# Autodesk Inventor assembly: Assembly3
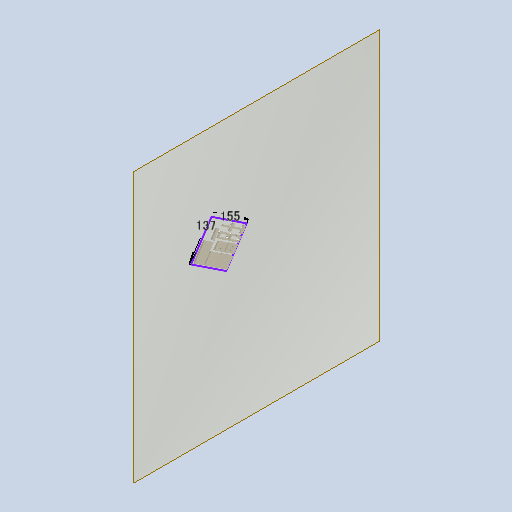
[picture p0: Inventor's stored thumbnail of the model, 512x512]
Saved by Autodesk Inventor 2025.1 (Build 291241000, 241)
## iProperties
Created: 2024-12-16
Part Number: Assembly3
Document SubType Name: Assembly
Designer: haruy
Author: haruy
## Documents named in this file (8)
- C:\Users\haruy\Documents\ロボコン\NHK2025\cad\cnc\Assembly3.iam
- C:\Users\haruy\Documents\ロボコン\NHK2025\cad\nagahisa\belt_liner\belt_liner_v1_Plate_6.ipt
- C:\Users\haruy\Documents\ロボコン\NHK2025\cad\nagahisa\belt_liner\belt_liner_v1_Plate_7.ipt
- C:\Users\haruy\Documents\ロボコン\NHK2025\cad\nagahisa\belt_liner\belt_liner_v1_Plate_9.ipt
- C:\Users\haruy\Documents\ロボコン\NHK2025\cad\nagahisa\belt_liner\belt_liner_v1_Plate_2.ipt
- C:\Users\haruy\Documents\ロボコン\NHK2025\cad\nagahisa\belt_liner\belt_liner_v1_Plate_1.ipt
- C:\Users\haruy\Documents\ロボコン\NHK2025\cad\nagahisa\belt_liner\belt_liner_v1_Plate_10.ipt
- C:\Users\haruy\Documents\ロボコン\NHK2025\cad\nagahisa\belt_liner\belt_liner_v1_Plate_15.ipt
## Components (9 placed, 7 different names)
1. belt_liner_v1_Plate_6:1 — フラッシュ:1, フラッシュ:5, メイト:1, メイト:2, フラッシュ:6, フラッシュ:8, メイト:4, フラッシュ:12
2. belt_liner_v1_Plate_7:1 — フラッシュ:2, フラッシュ:5, メイト:1
3. belt_liner_v1_Plate_9:1 — フラッシュ:4, メイト:2, フラッシュ:6, メイト:3, メイト:6
4. belt_liner_v1_Plate_9:2 — フラッシュ:3, メイト:3
5. belt_liner_v1_Plate_2:1 — フラッシュ:7, フラッシュ:8, メイト:4, フラッシュ:10, メイト:5
6. belt_liner_v1_Plate_1:1 — フラッシュ:9, フラッシュ:10, メイト:5, メイト:8, フラッシュ:16
7. belt_liner_v1_Plate_10:1 — フラッシュ:11, フラッシュ:12, メイト:6, メイト:7, フラッシュ:14
8. belt_liner_v1_Plate_10:2 — フラッシュ:13, メイト:7, フラッシュ:14
9. belt_liner_v1_Plate_15:1 — フラッシュ:15, メイト:8, フラッシュ:16
## Relationships (24: Flush 16, Mate 8)
- フラッシュ:1 [Flush]: belt_liner_v1_Plate_6:1
- フラッシュ:2 [Flush]: belt_liner_v1_Plate_7:1
- フラッシュ:3 [Flush]: belt_liner_v1_Plate_9:2
- フラッシュ:4 [Flush]: belt_liner_v1_Plate_9:1
- フラッシュ:5 [Flush]: belt_liner_v1_Plate_6:1 ↔ belt_liner_v1_Plate_7:1
- メイト:1 [Mate] (5 mm): belt_liner_v1_Plate_6:1 ↔ belt_liner_v1_Plate_7:1
- メイト:2 [Mate] (5 mm): belt_liner_v1_Plate_6:1 ↔ belt_liner_v1_Plate_9:1
- フラッシュ:6 [Flush]: belt_liner_v1_Plate_6:1 ↔ belt_liner_v1_Plate_9:1
- メイト:3 [Mate] (5 mm): belt_liner_v1_Plate_9:1 ↔ belt_liner_v1_Plate_9:2
- フラッシュ:7 [Flush]: belt_liner_v1_Plate_2:1
- フラッシュ:8 [Flush]: belt_liner_v1_Plate_6:1 ↔ belt_liner_v1_Plate_2:1
- メイト:4 [Mate] (5 mm): belt_liner_v1_Plate_6:1 ↔ belt_liner_v1_Plate_2:1
- フラッシュ:9 [Flush]: belt_liner_v1_Plate_1:1
- フラッシュ:10 [Flush]: belt_liner_v1_Plate_2:1 ↔ belt_liner_v1_Plate_1:1
- メイト:5 [Mate] (5 mm): belt_liner_v1_Plate_2:1 ↔ belt_liner_v1_Plate_1:1
- フラッシュ:11 [Flush]: belt_liner_v1_Plate_10:1
- フラッシュ:12 [Flush]: belt_liner_v1_Plate_6:1 ↔ belt_liner_v1_Plate_10:1
- メイト:6 [Mate] (5 mm): belt_liner_v1_Plate_9:1 ↔ belt_liner_v1_Plate_10:1
- フラッシュ:13 [Flush]: belt_liner_v1_Plate_10:2
- メイト:7 [Mate] (5 mm): belt_liner_v1_Plate_10:1 ↔ belt_liner_v1_Plate_10:2
- フラッシュ:14 [Flush]: belt_liner_v1_Plate_10:1 ↔ belt_liner_v1_Plate_10:2
- フラッシュ:15 [Flush]: belt_liner_v1_Plate_15:1
- メイト:8 [Mate] (5 mm): belt_liner_v1_Plate_1:1 ↔ belt_liner_v1_Plate_15:1
- フラッシュ:16 [Flush]: belt_liner_v1_Plate_1:1 ↔ belt_liner_v1_Plate_15:1
